# Autodesk Inventor assembly: ASSEMBLY_X_Axis_Carriage_and_Extruder_Belt_Gearbox
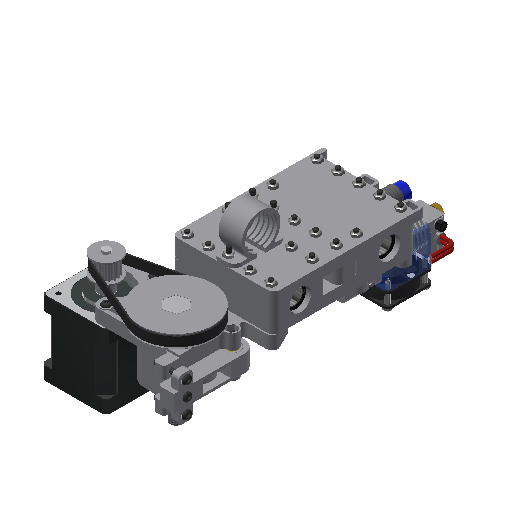
[picture p0: Inventor's stored thumbnail of the model, 512x512]
Saved by Autodesk Inventor 2026.1 (Build 301233000, 233)
## iProperties
Created: 2016-01-21
Part Number: ASSEMBLY_X_Axis_Carriage_and_Extruder_Belt_Gearbox
Material: Ogólny
Document SubType Name: Assembly
Designer: Andrzej
Author: Andrzej
## Documents named in this file (36)
- C:\Users\Andrzej\OneDrive\_DRIVE_SYNCH_FILES\__ BYTECHLAB PROJECTS\MECH - T-REX 300 – A completely new printer based on a old one\MCAD\1_REV1\ASSEMBLY_X_AXIS_CARRIAGE_AND_EXTRUDER\ASSEMBLY_X_Axis_Carriage_and_Extruder_Belt_Gearbox.iam
- C:\Users\Andrzej\OneDrive\_DRIVE_SYNCH_FILES\__ BYTECHLAB PROJECTS\MECH - T-REX 300 – A completely new printer based on a old one\MCAD\1_REV1\__COTS_PARTS\COTS_GENERIC_M8_Hobbed_Bolt.ipt
- C:\Users\Andrzej\OneDrive\_DRIVE_SYNCH_FILES\__ BYTECHLAB PROJECTS\MECH - T-REX 300 – A completely new printer based on a old one\MCAD\1_REV1\ASSEMBLY_X_AXIS_CARRIAGE_AND_EXTRUDER\3DP_ABS_HTD3M_Pulley_56_tooth_6mm.ipt
- C:\Users\Andrzej\OneDrive\_DRIVE_SYNCH_FILES\__ BYTECHLAB PROJECTS\MECH - T-REX 300 – A completely new printer based on a old one\MCAD\1_REV1\ASSEMBLY_X_AXIS_CARRIAGE_AND_EXTRUDER\3DP_ABS_X_Axis_Carriage_Front.ipt
- C:\Users\Andrzej\OneDrive\_DRIVE_SYNCH_FILES\__ BYTECHLAB PROJECTS\MECH - T-REX 300 – A completely new printer based on a old one\MCAD\1_REV1\ASSEMBLY_X_AXIS_CARRIAGE_AND_EXTRUDER\3DP_ABS_X_Axis_Carriage_Back.ipt
- C:\Users\Andrzej\OneDrive\_DRIVE_SYNCH_FILES\__ BYTECHLAB PROJECTS\MECH - T-REX 300 – A completely new printer based on a old one\MCAD\1_REV1\ASSEMBLY_X_AXIS_CARRIAGE_AND_EXTRUDER\3DP_ABS_Extruder_Body.ipt
- C:\Users\Andrzej\OneDrive\_DRIVE_SYNCH_FILES\__ BYTECHLAB PROJECTS\MECH - T-REX 300 – A completely new printer based on a old one\MCAD\1_REV1\ASSEMBLY_X_AXIS_CARRIAGE_AND_EXTRUDER\3DP_ABS_Extruder_Tensioning_Arm.ipt
- C:\Users\Andrzej\OneDrive\_DRIVE_SYNCH_FILES\__ BYTECHLAB PROJECTS\MECH - T-REX 300 – A completely new printer based on a old one\MCAD\1_REV1\ASSEMBLY_X_AXIS_CARRIAGE_AND_EXTRUDER\3DP_ABS_Extruder_Tensioning_Arm_Screw_Mount.ipt
- C:\Users\Andrzej\OneDrive\_DRIVE_SYNCH_FILES\__ BYTECHLAB PROJECTS\MECH - T-REX 300 – A completely new printer based on a old one\MCAD\1_REV1\ASSEMBLY_X_AXIS_CARRIAGE_AND_EXTRUDER\3DP_ABS_E3DV6_Mount.ipt
- C:\Users\Andrzej\OneDrive\_DRIVE_SYNCH_FILES\__ BYTECHLAB PROJECTS\MECH - T-REX 300 – A completely new printer based on a old one\MCAD\1_REV1\ASSEMBLY_X_AXIS_CARRIAGE_AND_EXTRUDER\CUT_PTFE_Tube_85mm.ipt
- C:\Users\Andrzej\OneDrive\_DRIVE_SYNCH_FILES\__ BYTECHLAB PROJECTS\MECH - T-REX 300 – A completely new printer based on a old one\MCAD\1_REV1\ASSEMBLY_X_AXIS_CARRIAGE_AND_EXTRUDER\3DP_ABS_Cable_Pipe_Mount.ipt
- C:\Users\Andrzej\OneDrive\_DRIVE_SYNCH_FILES\__ BYTECHLAB PROJECTS\MECH - T-REX 300 – A completely new printer based on a old one\MCAD\1_REV1\ASSEMBLY_X_AXIS_CARRIAGE_AND_EXTRUDER\3DP_ABS_PTFE_Tube_Stiffener.ipt
- C:\Users\Andrzej\OneDrive\_DRIVE_SYNCH_FILES\__ BYTECHLAB PROJECTS\MECH - T-REX 300 – A completely new printer based on a old one\MCAD\1_REV1\ASSEMBLY_X_AXIS_CARRIAGE_AND_EXTRUDER\3DP_ABS_E3DV6_Mounting_Clamp.ipt
- C:\Users\Andrzej\OneDrive\_DRIVE_SYNCH_FILES\__ BYTECHLAB PROJECTS\MECH - T-REX 300 – A completely new printer based on a old one\MCAD\1_REV1\__COTS_PARTS\COTS_E3D_V6_Hotend\COTS_E3D_V6_Hotend.iam
- C:\Users\Andrzej\OneDrive\_DRIVE_SYNCH_FILES\__ BYTECHLAB PROJECTS\MECH - T-REX 300 – A completely new printer based on a old one\MCAD\1_REV1\__COTS_PARTS\COTS_GENERIC_Induction_Distance_Sensor.ipt
- C:\Users\Andrzej\OneDrive\_DRIVE_SYNCH_FILES\__ BYTECHLAB PROJECTS\MECH - T-REX 300 – A completely new printer based on a old one\MCAD\1_REV1\ASSEMBLY_X_AXIS_CARRIAGE_AND_EXTRUDER\3DP_ABS_Induction_Sensor_Mount.ipt
- C:\Users\Andrzej\OneDrive\_DRIVE_SYNCH_FILES\__ BYTECHLAB PROJECTS\MECH - T-REX 300 – A completely new printer based on a old one\MCAD\1_REV1\ASSEMBLY_X_AXIS_CARRIAGE_AND_EXTRUDER\3DP_ABS_Induction_Sensor_Mounting_Clamp.ipt
- C:\Users\Andrzej\OneDrive\_DRIVE_SYNCH_FILES\__ BYTECHLAB PROJECTS\MECH - T-REX 300 – A completely new printer based on a old one\MCAD\1_REV1\ASSEMBLY_X_AXIS_CARRIAGE_AND_EXTRUDER\3DP_ABS_Induction_Sensor_Mount_Spacer.ipt
- C:\Users\Andrzej\OneDrive\_DRIVE_SYNCH_FILES\__ BYTECHLAB PROJECTS\MECH - T-REX 300 – A completely new printer based on a old one\MCAD\1_REV1\__COTS_PARTS\COTS_GENERIC_LM10UU_10mm_Linear_Bearing.ipt
- C:\Users\Andrzej\OneDrive\_DRIVE_SYNCH_FILES\__ BYTECHLAB PROJECTS\MECH - T-REX 300 – A completely new printer based on a old one\MCAD\1_REV1\__CONTENT_CENTER_PARTS\en-US\ISO 7380-1\ISO 7380-1 - M3 x 25.ipt
- C:\Users\Andrzej\OneDrive\_DRIVE_SYNCH_FILES\__ BYTECHLAB PROJECTS\MECH - T-REX 300 – A completely new printer based on a old one\MCAD\1_REV1\__CONTENT_CENTER_PARTS\en-US\DIN 934\DIN 934 - M3 x 0,5.ipt
- C:\Users\Andrzej\OneDrive\_DRIVE_SYNCH_FILES\__ BYTECHLAB PROJECTS\MECH - T-REX 300 – A completely new printer based on a old one\MCAD\1_REV1\__CONTENT_CENTER_PARTS\en-US\ISO 7380-1\ISO 7380-1 - M3 x 30.ipt
- C:\Users\Andrzej\OneDrive\_DRIVE_SYNCH_FILES\__ BYTECHLAB PROJECTS\MECH - T-REX 300 – A completely new printer based on a old one\MCAD\1_REV1\__CONTENT_CENTER_PARTS\en-US\ISO 7380-1\ISO 7380-1 - M3 x 20.ipt
- C:\Users\Andrzej\OneDrive\_DRIVE_SYNCH_FILES\__ BYTECHLAB PROJECTS\MECH - T-REX 300 – A completely new printer based on a old one\MCAD\1_REV1\__COTS_PARTS\COTS_GENERIC_ISO7380_M3x35.ipt
- C:\Users\Andrzej\OneDrive\_DRIVE_SYNCH_FILES\__ BYTECHLAB PROJECTS\MECH - T-REX 300 – A completely new printer based on a old one\MCAD\1_REV1\__COTS_PARTS\COTS_GENERIC_ISO7380_M3x45.ipt
- C:\Users\Andrzej\OneDrive\_DRIVE_SYNCH_FILES\__ BYTECHLAB PROJECTS\MECH - T-REX 300 – A completely new printer based on a old one\MCAD\1_REV1\__CONTENT_CENTER_PARTS\en-US\DIN 125-1  A\DIN 125 - A 3,2.ipt
- C:\Users\Andrzej\OneDrive\_DRIVE_SYNCH_FILES\__ BYTECHLAB PROJECTS\MECH - T-REX 300 – A completely new printer based on a old one\MCAD\1_REV1\__CONTENT_CENTER_PARTS\en-US\ISO 7380-1\ISO 7380-1 - M3 x 12.ipt
- C:\Users\Andrzej\OneDrive\_DRIVE_SYNCH_FILES\__ BYTECHLAB PROJECTS\MECH - T-REX 300 – A completely new printer based on a old one\MCAD\1_REV1\__CONTENT_CENTER_PARTS\en-US\DIN 934\DIN 934 - M8 x 1,25.ipt
- C:\Users\Andrzej\OneDrive\_DRIVE_SYNCH_FILES\__ BYTECHLAB PROJECTS\MECH - T-REX 300 – A completely new printer based on a old one\MCAD\1_REV1\__COTS_PARTS\COTS_GENERIC_608_2RS_8x22x7mm_bearing.ipt
- C:\Users\Andrzej\OneDrive\_DRIVE_SYNCH_FILES\__ BYTECHLAB PROJECTS\MECH - T-REX 300 – A completely new printer based on a old one\MCAD\1_REV1\__COTS_PARTS\COTS_GENERIC_623_ZZ_3x10x4mm_bearing\COTS_GENERIC_623_ZZ_3x10x4mm_bearing.ipt
- C:\Users\Andrzej\OneDrive\_DRIVE_SYNCH_FILES\__ BYTECHLAB PROJECTS\MECH - T-REX 300 – A completely new printer based on a old one\MCAD\1_REV1\__COTS_PARTS\COTS_Optibelt_Omega_HTD3M_204T_6mm.ipt
- C:\Users\Andrzej\OneDrive\_DRIVE_SYNCH_FILES\__ BYTECHLAB PROJECTS\MECH - T-REX 300 – A completely new printer based on a old one\MCAD\1_REV1\__COTS_PARTS\COTS_UNKNOWN_HTD3M_16T_Pulley\COTS_UNKNOWN_HTD3M_16T_Pulley.ipt
- C:\Users\Andrzej\OneDrive\_DRIVE_SYNCH_FILES\__ BYTECHLAB PROJECTS\MECH - T-REX 300 – A completely new printer based on a old one\MCAD\1_REV1\__COTS_PARTS\COTS_GENERIC_635_HZZ_5x19x6mm_bearing\COTS_GENERIC_635_HZZ_5x19x6mm_bearing.ipt
- C:\Users\Andrzej\OneDrive\_DRIVE_SYNCH_FILES\__ BYTECHLAB PROJECTS\MECH - T-REX 300 – A completely new printer based on a old one\MCAD\1_REV1\ASSEMBLY_X_AXIS_CARRIAGE_AND_EXTRUDER\CUT_STEEL_5x11mm_Rod.ipt
- C:\Users\Andrzej\OneDrive\_DRIVE_SYNCH_FILES\__ BYTECHLAB PROJECTS\MECH - T-REX 300 – A completely new printer based on a old one\MCAD\1_REV1\__COTS_PARTS\COTS_GENERIC_NEMA17_25mm_shaft.ipt
- C:\Users\Andrzej\OneDrive\_DRIVE_SYNCH_FILES\__ BYTECHLAB PROJECTS\MECH - T-REX 300 – A completely new printer based on a old one\MCAD\1_REV1\ASSEMBLY_X_AXIS_CARRIAGE_AND_EXTRUDER\3DP_ABS_Hobbed_Bolt_Spacer.ipt
## Components (100 placed, 35 different names)
1. 3DP_ABS_X_Axis_Carriage_Front:1 — Zestawiający:1, Równoległy:1, Równoległy:2, Zestawiający:2, Styczny:1, Zestawiający:19, Zestawiający:28, Mate:33, Mate:34, Mate:35, Mate:43, Mate:44, Mate:45, Mate:46, Mate:49, Mate:50, Mate:65, Mate:108, Mate:109, Mate:110, Mate:111, Mate:112, Mate:113, Mate:114, Mate:115, Mate:116, Mate:117, Mate:118, Mate:119, Mate:120, Mate:122, Mate:124, Mate:126, Mate:128, Mate:130, Mate:134, Mate:135, Mate:136
2. 3DP_ABS_X_Axis_Carriage_Back:1 — Zestawiający:1, Równoległy:1, Równoległy:2, Zestawiający:27, Mate:70, Mate:72, Mate:75, Mate:77, Mate:78, Mate:79, Mate:80, Mate:81, Mate:99, Mate:101, Mate:103, Mate:105, Mate:106, Mate:107, Mate:121, Mate:123, Mate:125, Mate:127, Mate:129, Mate:131, Mate:143, Mate:145, Insert:3, Insert:4, Insert:5, Insert:6
3. 3DP_ABS_Extruder_Body:1 — Zestawiający:2, Styczny:1, Zestawiający:4, Styczny:4, Zestawiający:6, Równoległy:3, Zestawiający:8, Wstaw:1, Mate:51, Mate:52, Mate:55, Mate:56, Mate:90, Mate:91, Mate:92, Mate:93, Mate:94, Mate:95, Mate:96, Mate:97, Mate:98, Mate:100, Mate:102, Mate:104, Mate:132, Mate:133, Mate:155, Mate:157, Mate:159, Mate:168, Mate:169, Mate:170, Mate:171, Angle:3, Mate:180, Mate:182, Mate:184, Mate:185, Mate:186, Mate:187
4. 3DP_ABS_HTD3M_Pulley_56_tooth_6mm:1 — Zestawiający:3, Styczny:2, Zestawiający:4, Angle:2, Mate:173, Mate:174, Mate:176
5. COTS_GENERIC_M8_Hobbed_Bolt:1 — Zestawiający:3, Styczny:2, Mate:53, Angle:2, Mate:188
6. COTS_GENERIC_NEMA17_25mm_shaft:1 — Zestawiający:6, Równoległy:3, Mate:154, Mate:156, Mate:158, Mate:172
7. 3DP_ABS_Extruder_Tensioning_Arm:1 — Styczny:4, Zestawiający:8, Zestawiający:9, Zestawiający:10, Równoległy:4, Mate:163, Mate:164, Mate:165, Mate:166, Mate:167, Mate:177, Mate:178, Mate:179, Flush:16
8. 3DP_ABS_Extruder_Tensioning_Arm_Screw_Mount:1 — Zestawiający:9, Zestawiający:10, Równoległy:4, Mate:160, Mate:161, Mate:162, Angle:3, Mate:181, Mate:183
9. 3DP_ABS_E3DV6_Mount:1 — Zestawiający:19, Zestawiający:30, Zestawiający:31, Zestawiający:32, Równoległy:13, Równoległy:14, Mate:57, Mate:58, Mate:60, Mate:61, Mate:65, Mate:66, Mate:67, Mate:68, Mate:69, Mate:71, Mate:73, Mate:74, Mate:76
10. CUT_PTFE_Tube_85mm:1 — Wstaw:1, Zestawiający:29
11. 3DP_ABS_Cable_Pipe_Mount:1 — Zestawiający:27, Mate:106, Mate:107, Insert:2, Mate:137
12. 3DP_ABS_PTFE_Tube_Stiffener:1 — Zestawiający:28, Zestawiający:29, Mate:138, Mate:139, Mate:140, Mate:141, Mate:142, Mate:144
13. 3DP_ABS_E3DV6_Mounting_Clamp:1 — Zestawiający:32, Równoległy:13, Równoległy:14, Mate:59, Mate:62, Mate:63, Mate:64
14. COTS_E3D_V6_Hotend:1 [sub-assembly] — Zestawiający:30, Zestawiający:31, Flush:15
15. COTS_GENERIC_Induction_Distance_Sensor:1 — Mate:40, Flush:15, Mate:41
16. 3DP_ABS_Induction_Sensor_Mount:1 — Mate:36, Mate:37, Mate:38, Mate:39, Mate:40, Angle:1, Mate:42, Mate:87, Mate:89, Mate:146, Mate:147, Mate:148, Mate:149, Mate:150, Mate:151, Mate:152, Mate:153
17. 3DP_ABS_Induction_Sensor_Mounting_Clamp:1 — Mate:41, Angle:1, Mate:42, Mate:82, Mate:83, Mate:84, Mate:85, Mate:86, Mate:88
18. 3DP_ABS_Induction_Sensor_Mount_Spacer:1 — Mate:33, Mate:34, Mate:35, Mate:36, Mate:37, Mate:38, Mate:39
19. COTS_GENERIC_LM10UU_10mm_Linear_Bearing:1 — Mate:45, Mate:48, Mate:49
20. COTS_GENERIC_LM10UU_10mm_Linear_Bearing:2 — Mate:46, Mate:48
21. COTS_GENERIC_LM10UU_10mm_Linear_Bearing:3 — Mate:44, Mate:47, Mate:50
22. COTS_GENERIC_LM10UU_10mm_Linear_Bearing:4 — Mate:43, Mate:47
23. COTS_GENERIC_608_2RS_8x22x7mm_bearing:1 — Mate:55, Mate:56, Mate:189
24. COTS_GENERIC_608_2RS_8x22x7mm_bearing:2 — Mate:51, Mate:52, Mate:53, Insert:10
25. COTS_GENERIC_623_ZZ_3x10x4mm_bearing:1 — Mate:165, Mate:166, Insert:12
26. COTS_GENERIC_623_ZZ_3x10x4mm_bearing:2 — Mate:164, Mate:167, Insert:11
27. COTS_Optibelt_Omega_HTD3M_204T_6mm:1 — Mate:174, Mate:175, Mate:176
28. COTS_UNKNOWN_HTD3M_16T_Pulley:1 — Mate:172, Mate:173, Mate:175
29. COTS_GENERIC_635_HZZ_5x19x6mm_bearing:1 — Mate:177, Mate:178
30. CUT_STEEL_5x11mm_Rod:1 — Mate:179, Flush:16
31. 3DP_ABS_Hobbed_Bolt_Spacer:1 — Mate:188, Mate:189
32. DIN 934 - replaced by DIN EN 24032/28673/28674 M3:30 — Mate:186, Mate:187
33. ISO 7380-1 M3 x 20:4 — Mate:182, Mate:183
34. DIN 934 - replaced by DIN EN 24032/28673/28674 M3:29 — Mate:184, Mate:185
35. ISO 7380-1 M3 x 20:3 — Mate:180, Mate:181
36. DIN 934 - replaced by DIN EN 24032/28673/28674 M3:28 — Mate:170, Mate:171
37. ISO 7380-1 M3 x 25:9 — Mate:168, Mate:169
38. DIN 125-1 A A 3,2:5 — Insert:12
39. DIN 125-1 A A 3,2:4 — Insert:11
40. DIN 934 - replaced by DIN EN 24032/28673/28674 M3:27 — Mate:162, Mate:163
41. ISO 7380-1 M3 x 12:4 — Mate:160, Mate:161
42. DIN 934 - replaced by DIN EN 24032/28673/28674 M8:1 — Insert:10
43. ISO 7380-1 M3 x 12:3 — Insert:9
44. ISO 7380-1 M3 x 12:2 — Insert:8
45. DIN 125-1 A A 3,2:3 — Mate:158, Mate:159, Insert:9
46. DIN 125-1 A A 3,2:2 — Mate:156, Mate:157, Insert:8
47. ISO 7380-1 M3 x 12:1 — Insert:7
48. DIN 125-1 A A 3,2:1 — Mate:154, Mate:155, Insert:7
49. DIN 934 - replaced by DIN EN 24032/28673/28674 M3:26 — Insert:6
50. DIN 934 - replaced by DIN EN 24032/28673/28674 M3:25 — Insert:5
51. DIN 934 - replaced by DIN EN 24032/28673/28674 M3:24 — Insert:4
52. DIN 934 - replaced by DIN EN 24032/28673/28674 M3:23 — Insert:3
53. COTS_GENERIC_ISO7380_M3x45:4 — Mate:148, Mate:153
54. COTS_GENERIC_ISO7380_M3x45:3 — Mate:149, Mate:151
55. COTS_GENERIC_ISO7380_M3x45:2 — Mate:147, Mate:152
56. COTS_GENERIC_ISO7380_M3x45:1 — Mate:146, Mate:150
57. DIN 934 - replaced by DIN EN 24032/28673/28674 M3:22 — Mate:144, Mate:145
58. ISO 7380-1 M3 x 30:11 — Mate:140, Mate:141
59. DIN 934 - replaced by DIN EN 24032/28673/28674 M3:21 — Mate:142, Mate:143
60. ISO 7380-1 M3 x 30:10 — Mate:138, Mate:139
61. DIN 934 - replaced by DIN EN 24032/28673/28674 M3:20 — Mate:136, Mate:137
62. ISO 7380-1 M3 x 30:9 — Mate:134, Mate:135
63. DIN 934 - replaced by DIN EN 24032/28673/28674 M3:19 — Insert:2
64. COTS_GENERIC_ISO7380_M3x35:2 — Mate:132, Mate:133
65. DIN 934 - replaced by DIN EN 24032/28673/28674 M3:18 — Mate:130, Mate:131
66. DIN 934 - replaced by DIN EN 24032/28673/28674 M3:17 — Mate:128, Mate:129
67. DIN 934 - replaced by DIN EN 24032/28673/28674 M3:16 — Mate:126, Mate:127
68. DIN 934 - replaced by DIN EN 24032/28673/28674 M3:15 — Mate:124, Mate:125
69. DIN 934 - replaced by DIN EN 24032/28673/28674 M3:14 — Mate:122, Mate:123
70. ISO 7380-1 M3 x 25:8 — Mate:118, Mate:119
71. ISO 7380-1 M3 x 25:7 — Mate:116, Mate:117
72. ISO 7380-1 M3 x 25:6 — Mate:114, Mate:115
73. ISO 7380-1 M3 x 25:5 — Mate:112, Mate:113
74. ISO 7380-1 M3 x 25:4 — Mate:110, Mate:111
75. DIN 934 - replaced by DIN EN 24032/28673/28674 M3:13 — Mate:120, Mate:121
76. ISO 7380-1 M3 x 25:3 — Mate:108, Mate:109
77. DIN 934 - replaced by DIN EN 24032/28673/28674 M3:12 — Mate:104, Mate:105
78. DIN 934 - replaced by DIN EN 24032/28673/28674 M3:11 — Mate:102, Mate:103
79. DIN 934 - replaced by DIN EN 24032/28673/28674 M3:10 — Mate:100, Mate:101
80. ISO 7380-1 M3 x 30:8 — Mate:96, Mate:97
81. ISO 7380-1 M3 x 30:7 — Mate:94, Mate:95
82. ISO 7380-1 M3 x 30:6 — Mate:92, Mate:93
83. DIN 934 - replaced by DIN EN 24032/28673/28674 M3:9 — Mate:98, Mate:99
84. ISO 7380-1 M3 x 30:5 — Mate:90, Mate:91
85. DIN 934 - replaced by DIN EN 24032/28673/28674 M3:8 — Mate:88, Mate:89
86. ISO 7380-1 M3 x 20:2 — Mate:84, Mate:85
87. DIN 934 - replaced by DIN EN 24032/28673/28674 M3:7 — Mate:86, Mate:87
88. ISO 7380-1 M3 x 20:1 — Mate:82, Mate:83
89. DIN 934 - replaced by DIN EN 24032/28673/28674 M3:6 — Mate:80, Mate:81
90. DIN 934 - replaced by DIN EN 24032/28673/28674 M3:5 — Mate:78, Mate:79
91. DIN 934 - replaced by DIN EN 24032/28673/28674 M3:4 — Mate:76, Mate:77
92. ISO 7380-1 M3 x 30:4 — Mate:72, Mate:73
93. ISO 7380-1 M3 x 30:3 — Mate:70, Mate:71
94. ISO 7380-1 M3 x 30:2 — Mate:68, Mate:69
95. DIN 934 - replaced by DIN EN 24032/28673/28674 M3:3 — Mate:74, Mate:75
96. ISO 7380-1 M3 x 30:1 — Mate:66, Mate:67
97. DIN 934 - replaced by DIN EN 24032/28673/28674 M3:2 — Mate:63, Mate:64
98. ISO 7380-1 M3 x 25:2 — Mate:59, Mate:60
99. DIN 934 - replaced by DIN EN 24032/28673/28674 M3:1 — Mate:61, Mate:62
100. ISO 7380-1 M3 x 25:1 — Mate:57, Mate:58
## Relationships (197: Mate 171, Insert 12, Flush 8, Tangent 3, Angle 3)
- Zestawiający:1 [Mate]: 3DP_ABS_X_Axis_Carriage_Front:1 ↔ 3DP_ABS_X_Axis_Carriage_Back:1
- Równoległy:1 [Flush]: 3DP_ABS_X_Axis_Carriage_Front:1 ↔ 3DP_ABS_X_Axis_Carriage_Back:1
- Równoległy:2 [Flush]: 3DP_ABS_X_Axis_Carriage_Front:1 ↔ 3DP_ABS_X_Axis_Carriage_Back:1
- Zestawiający:2 [Mate]: 3DP_ABS_X_Axis_Carriage_Front:1 ↔ 3DP_ABS_Extruder_Body:1
- Styczny:1 [Tangent]: 3DP_ABS_X_Axis_Carriage_Front:1 ↔ 3DP_ABS_Extruder_Body:1
- Zestawiający:3 [Mate]: 3DP_ABS_HTD3M_Pulley_56_tooth_6mm:1 ↔ COTS_GENERIC_M8_Hobbed_Bolt:1
- Styczny:2 [Tangent]: 3DP_ABS_HTD3M_Pulley_56_tooth_6mm:1 ↔ COTS_GENERIC_M8_Hobbed_Bolt:1
- Zestawiający:4 [Mate] (4 mm): 3DP_ABS_Extruder_Body:1 ↔ 3DP_ABS_HTD3M_Pulley_56_tooth_6mm:1
- Styczny:4 [Tangent]: 3DP_ABS_Extruder_Body:1 ↔ 3DP_ABS_Extruder_Tensioning_Arm:1
- Zestawiający:6 [Mate]: 3DP_ABS_Extruder_Body:1 ↔ COTS_GENERIC_NEMA17_25mm_shaft:1
- Równoległy:3 [Flush] (-1.5 mm): 3DP_ABS_Extruder_Body:1 ↔ COTS_GENERIC_NEMA17_25mm_shaft:1
- Zestawiający:8 [Mate] (0.5 mm): 3DP_ABS_Extruder_Body:1 ↔ 3DP_ABS_Extruder_Tensioning_Arm:1
- Zestawiający:9 [Mate]: 3DP_ABS_Extruder_Tensioning_Arm:1 ↔ 3DP_ABS_Extruder_Tensioning_Arm_Screw_Mount:1
- Zestawiający:10 [Mate]: 3DP_ABS_Extruder_Tensioning_Arm:1 ↔ 3DP_ABS_Extruder_Tensioning_Arm_Screw_Mount:1
- Równoległy:4 [Flush]: 3DP_ABS_Extruder_Tensioning_Arm:1 ↔ 3DP_ABS_Extruder_Tensioning_Arm_Screw_Mount:1
- Zestawiający:19 [Mate]: 3DP_ABS_X_Axis_Carriage_Front:1 ↔ 3DP_ABS_E3DV6_Mount:1
- Wstaw:1 [Insert]: 3DP_ABS_Extruder_Body:1 ↔ CUT_PTFE_Tube_85mm:1
- Zestawiający:27 [Mate]: 3DP_ABS_X_Axis_Carriage_Back:1 ↔ 3DP_ABS_Cable_Pipe_Mount:1
- Zestawiający:28 [Mate]: 3DP_ABS_X_Axis_Carriage_Front:1 ↔ 3DP_ABS_PTFE_Tube_Stiffener:1
- Zestawiający:29 [Mate]: CUT_PTFE_Tube_85mm:1 ↔ 3DP_ABS_PTFE_Tube_Stiffener:1
- Zestawiający:30 [Mate]: 3DP_ABS_E3DV6_Mount:1 ↔ COTS_E3D_V6_Hotend:1
- Zestawiający:31 [Mate] (0.2 mm): 3DP_ABS_E3DV6_Mount:1 ↔ COTS_E3D_V6_Hotend:1
- Zestawiający:32 [Mate]: 3DP_ABS_E3DV6_Mount:1 ↔ 3DP_ABS_E3DV6_Mounting_Clamp:1
- Równoległy:13 [Flush]: 3DP_ABS_E3DV6_Mount:1 ↔ 3DP_ABS_E3DV6_Mounting_Clamp:1
- Równoległy:14 [Flush]: 3DP_ABS_E3DV6_Mount:1 ↔ 3DP_ABS_E3DV6_Mounting_Clamp:1
- Mate:33: 3DP_ABS_X_Axis_Carriage_Front:1 ↔ 3DP_ABS_Induction_Sensor_Mount_Spacer:1
- Mate:34: 3DP_ABS_X_Axis_Carriage_Front:1 ↔ 3DP_ABS_Induction_Sensor_Mount_Spacer:1
- Mate:35: 3DP_ABS_X_Axis_Carriage_Front:1 ↔ 3DP_ABS_Induction_Sensor_Mount_Spacer:1
- Mate:36: 3DP_ABS_Induction_Sensor_Mount:1 ↔ 3DP_ABS_Induction_Sensor_Mount_Spacer:1
- Mate:37: 3DP_ABS_Induction_Sensor_Mount:1 ↔ 3DP_ABS_Induction_Sensor_Mount_Spacer:1
- Mate:38: 3DP_ABS_Induction_Sensor_Mount:1 ↔ 3DP_ABS_Induction_Sensor_Mount_Spacer:1
- Mate:39: 3DP_ABS_Induction_Sensor_Mount:1 ↔ 3DP_ABS_Induction_Sensor_Mount_Spacer:1
- Mate:40: COTS_GENERIC_Induction_Distance_Sensor:1 ↔ 3DP_ABS_Induction_Sensor_Mount:1
- Flush:15 (2 mm): COTS_E3D_V6_Hotend:1 ↔ COTS_GENERIC_Induction_Distance_Sensor:1
- Mate:41: COTS_GENERIC_Induction_Distance_Sensor:1 ↔ 3DP_ABS_Induction_Sensor_Mounting_Clamp:1
- Angle:1 (0 deg): 3DP_ABS_Induction_Sensor_Mount:1 ↔ 3DP_ABS_Induction_Sensor_Mounting_Clamp:1
- Mate:42: 3DP_ABS_Induction_Sensor_Mount:1 ↔ 3DP_ABS_Induction_Sensor_Mounting_Clamp:1
- Mate:43: 3DP_ABS_X_Axis_Carriage_Front:1 ↔ COTS_GENERIC_LM10UU_10mm_Linear_Bearing:4
- Mate:44: 3DP_ABS_X_Axis_Carriage_Front:1 ↔ COTS_GENERIC_LM10UU_10mm_Linear_Bearing:3
- Mate:45: 3DP_ABS_X_Axis_Carriage_Front:1 ↔ COTS_GENERIC_LM10UU_10mm_Linear_Bearing:1
- Mate:46: 3DP_ABS_X_Axis_Carriage_Front:1 ↔ COTS_GENERIC_LM10UU_10mm_Linear_Bearing:2
- Mate:47: COTS_GENERIC_LM10UU_10mm_Linear_Bearing:3 ↔ COTS_GENERIC_LM10UU_10mm_Linear_Bearing:4
- Mate:48: COTS_GENERIC_LM10UU_10mm_Linear_Bearing:1 ↔ COTS_GENERIC_LM10UU_10mm_Linear_Bearing:2
- Mate:49 (0.7 mm): 3DP_ABS_X_Axis_Carriage_Front:1 ↔ COTS_GENERIC_LM10UU_10mm_Linear_Bearing:1
- Mate:50 (0.7 mm): 3DP_ABS_X_Axis_Carriage_Front:1 ↔ COTS_GENERIC_LM10UU_10mm_Linear_Bearing:3
- Mate:51: 3DP_ABS_Extruder_Body:1 ↔ COTS_GENERIC_608_2RS_8x22x7mm_bearing:2
- Mate:52: 3DP_ABS_Extruder_Body:1 ↔ COTS_GENERIC_608_2RS_8x22x7mm_bearing:2
- Mate:53: COTS_GENERIC_M8_Hobbed_Bolt:1 ↔ COTS_GENERIC_608_2RS_8x22x7mm_bearing:2
- Mate:55: 3DP_ABS_Extruder_Body:1 ↔ COTS_GENERIC_608_2RS_8x22x7mm_bearing:1
- Mate:56: 3DP_ABS_Extruder_Body:1 ↔ COTS_GENERIC_608_2RS_8x22x7mm_bearing:1
- Angle:2 (0 deg): 3DP_ABS_HTD3M_Pulley_56_tooth_6mm:1 ↔ COTS_GENERIC_M8_Hobbed_Bolt:1
- Mate:57: 3DP_ABS_E3DV6_Mount:1 ↔ ISO 7380-1 M3 x 25:1
- Mate:58: 3DP_ABS_E3DV6_Mount:1 ↔ ISO 7380-1 M3 x 25:1
- Mate:59: 3DP_ABS_E3DV6_Mounting_Clamp:1 ↔ ISO 7380-1 M3 x 25:2
- Mate:60: 3DP_ABS_E3DV6_Mount:1 ↔ ISO 7380-1 M3 x 25:2
- Mate:61: 3DP_ABS_E3DV6_Mount:1 ↔ DIN 934 - replaced by DIN EN 24032/28673/28674 M3:1
- Mate:62: 3DP_ABS_E3DV6_Mounting_Clamp:1 ↔ DIN 934 - replaced by DIN EN 24032/28673/28674 M3:1
- Mate:63: 3DP_ABS_E3DV6_Mounting_Clamp:1 ↔ DIN 934 - replaced by DIN EN 24032/28673/28674 M3:2
- Mate:64: 3DP_ABS_E3DV6_Mounting_Clamp:1 ↔ DIN 934 - replaced by DIN EN 24032/28673/28674 M3:2
- Mate:65: 3DP_ABS_X_Axis_Carriage_Front:1 ↔ 3DP_ABS_E3DV6_Mount:1
- Mate:66: 3DP_ABS_E3DV6_Mount:1 ↔ ISO 7380-1 M3 x 30:1
- Mate:67: 3DP_ABS_E3DV6_Mount:1 ↔ ISO 7380-1 M3 x 30:1
- Mate:68: 3DP_ABS_E3DV6_Mount:1 ↔ ISO 7380-1 M3 x 30:2
- Mate:69: 3DP_ABS_E3DV6_Mount:1 ↔ ISO 7380-1 M3 x 30:2
- Mate:70: 3DP_ABS_X_Axis_Carriage_Back:1 ↔ ISO 7380-1 M3 x 30:3
- Mate:71: 3DP_ABS_E3DV6_Mount:1 ↔ ISO 7380-1 M3 x 30:3
- Mate:72: 3DP_ABS_X_Axis_Carriage_Back:1 ↔ ISO 7380-1 M3 x 30:4
- Mate:73: 3DP_ABS_E3DV6_Mount:1 ↔ ISO 7380-1 M3 x 30:4
- Mate:74: 3DP_ABS_E3DV6_Mount:1 ↔ DIN 934 - replaced by DIN EN 24032/28673/28674 M3:3
- Mate:75: 3DP_ABS_X_Axis_Carriage_Back:1 ↔ DIN 934 - replaced by DIN EN 24032/28673/28674 M3:3
- Mate:76: 3DP_ABS_E3DV6_Mount:1 ↔ DIN 934 - replaced by DIN EN 24032/28673/28674 M3:4
- Mate:77: 3DP_ABS_X_Axis_Carriage_Back:1 ↔ DIN 934 - replaced by DIN EN 24032/28673/28674 M3:4
- Mate:78: 3DP_ABS_X_Axis_Carriage_Back:1 ↔ DIN 934 - replaced by DIN EN 24032/28673/28674 M3:5
- Mate:79: 3DP_ABS_X_Axis_Carriage_Back:1 ↔ DIN 934 - replaced by DIN EN 24032/28673/28674 M3:5
- Mate:80: 3DP_ABS_X_Axis_Carriage_Back:1 ↔ DIN 934 - replaced by DIN EN 24032/28673/28674 M3:6
- Mate:81: 3DP_ABS_X_Axis_Carriage_Back:1 ↔ DIN 934 - replaced by DIN EN 24032/28673/28674 M3:6
- Mate:82: 3DP_ABS_Induction_Sensor_Mounting_Clamp:1 ↔ ISO 7380-1 M3 x 20:1
- Mate:83: 3DP_ABS_Induction_Sensor_Mounting_Clamp:1 ↔ ISO 7380-1 M3 x 20:1
- Mate:84: 3DP_ABS_Induction_Sensor_Mounting_Clamp:1 ↔ ISO 7380-1 M3 x 20:2
- Mate:85: 3DP_ABS_Induction_Sensor_Mounting_Clamp:1 ↔ ISO 7380-1 M3 x 20:2
- Mate:86: 3DP_ABS_Induction_Sensor_Mounting_Clamp:1 ↔ DIN 934 - replaced by DIN EN 24032/28673/28674 M3:7
- Mate:87: 3DP_ABS_Induction_Sensor_Mount:1 ↔ DIN 934 - replaced by DIN EN 24032/28673/28674 M3:7
- Mate:88: 3DP_ABS_Induction_Sensor_Mounting_Clamp:1 ↔ DIN 934 - replaced by DIN EN 24032/28673/28674 M3:8
- Mate:89: 3DP_ABS_Induction_Sensor_Mount:1 ↔ DIN 934 - replaced by DIN EN 24032/28673/28674 M3:8
- Mate:90: 3DP_ABS_Extruder_Body:1 ↔ ISO 7380-1 M3 x 30:5
- Mate:91: 3DP_ABS_Extruder_Body:1 ↔ ISO 7380-1 M3 x 30:5
- Mate:92: 3DP_ABS_Extruder_Body:1 ↔ ISO 7380-1 M3 x 30:6
- Mate:93: 3DP_ABS_Extruder_Body:1 ↔ ISO 7380-1 M3 x 30:6
- Mate:94: 3DP_ABS_Extruder_Body:1 ↔ ISO 7380-1 M3 x 30:7
- Mate:95: 3DP_ABS_Extruder_Body:1 ↔ ISO 7380-1 M3 x 30:7
- Mate:96: 3DP_ABS_Extruder_Body:1 ↔ ISO 7380-1 M3 x 30:8
- Mate:97: 3DP_ABS_Extruder_Body:1 ↔ ISO 7380-1 M3 x 30:8
- Mate:98: 3DP_ABS_Extruder_Body:1 ↔ DIN 934 - replaced by DIN EN 24032/28673/28674 M3:9
- Mate:99: 3DP_ABS_X_Axis_Carriage_Back:1 ↔ DIN 934 - replaced by DIN EN 24032/28673/28674 M3:9
- Mate:100: 3DP_ABS_Extruder_Body:1 ↔ DIN 934 - replaced by DIN EN 24032/28673/28674 M3:10
- Mate:101: 3DP_ABS_X_Axis_Carriage_Back:1 ↔ DIN 934 - replaced by DIN EN 24032/28673/28674 M3:10
- Mate:102: 3DP_ABS_Extruder_Body:1 ↔ DIN 934 - replaced by DIN EN 24032/28673/28674 M3:11
- Mate:103: 3DP_ABS_X_Axis_Carriage_Back:1 ↔ DIN 934 - replaced by DIN EN 24032/28673/28674 M3:11
- Mate:104: 3DP_ABS_Extruder_Body:1 ↔ DIN 934 - replaced by DIN EN 24032/28673/28674 M3:12
- Mate:105: 3DP_ABS_X_Axis_Carriage_Back:1 ↔ DIN 934 - replaced by DIN EN 24032/28673/28674 M3:12
- Mate:106: 3DP_ABS_X_Axis_Carriage_Back:1 ↔ 3DP_ABS_Cable_Pipe_Mount:1
- Mate:107: 3DP_ABS_X_Axis_Carriage_Back:1 ↔ 3DP_ABS_Cable_Pipe_Mount:1
- Mate:108: 3DP_ABS_X_Axis_Carriage_Front:1 ↔ ISO 7380-1 M3 x 25:3
- Mate:109: 3DP_ABS_X_Axis_Carriage_Front:1 ↔ ISO 7380-1 M3 x 25:3
- Mate:110: 3DP_ABS_X_Axis_Carriage_Front:1 ↔ ISO 7380-1 M3 x 25:4
- Mate:111: 3DP_ABS_X_Axis_Carriage_Front:1 ↔ ISO 7380-1 M3 x 25:4
- Mate:112: 3DP_ABS_X_Axis_Carriage_Front:1 ↔ ISO 7380-1 M3 x 25:5
- Mate:113: 3DP_ABS_X_Axis_Carriage_Front:1 ↔ ISO 7380-1 M3 x 25:5
- Mate:114: 3DP_ABS_X_Axis_Carriage_Front:1 ↔ ISO 7380-1 M3 x 25:6
- Mate:115: 3DP_ABS_X_Axis_Carriage_Front:1 ↔ ISO 7380-1 M3 x 25:6
- Mate:116: 3DP_ABS_X_Axis_Carriage_Front:1 ↔ ISO 7380-1 M3 x 25:7
- Mate:117: 3DP_ABS_X_Axis_Carriage_Front:1 ↔ ISO 7380-1 M3 x 25:7
- Mate:118: 3DP_ABS_X_Axis_Carriage_Front:1 ↔ ISO 7380-1 M3 x 25:8
- Mate:119: 3DP_ABS_X_Axis_Carriage_Front:1 ↔ ISO 7380-1 M3 x 25:8
- Mate:120: 3DP_ABS_X_Axis_Carriage_Front:1 ↔ DIN 934 - replaced by DIN EN 24032/28673/28674 M3:13
- Mate:121: 3DP_ABS_X_Axis_Carriage_Back:1 ↔ DIN 934 - replaced by DIN EN 24032/28673/28674 M3:13
- Mate:122: 3DP_ABS_X_Axis_Carriage_Front:1 ↔ DIN 934 - replaced by DIN EN 24032/28673/28674 M3:14
- Mate:123: 3DP_ABS_X_Axis_Carriage_Back:1 ↔ DIN 934 - replaced by DIN EN 24032/28673/28674 M3:14
- Mate:124: 3DP_ABS_X_Axis_Carriage_Front:1 ↔ DIN 934 - replaced by DIN EN 24032/28673/28674 M3:15
- Mate:125: 3DP_ABS_X_Axis_Carriage_Back:1 ↔ DIN 934 - replaced by DIN EN 24032/28673/28674 M3:15
- Mate:126: 3DP_ABS_X_Axis_Carriage_Front:1 ↔ DIN 934 - replaced by DIN EN 24032/28673/28674 M3:16
- Mate:127: 3DP_ABS_X_Axis_Carriage_Back:1 ↔ DIN 934 - replaced by DIN EN 24032/28673/28674 M3:16
- Mate:128: 3DP_ABS_X_Axis_Carriage_Front:1 ↔ DIN 934 - replaced by DIN EN 24032/28673/28674 M3:17
- Mate:129: 3DP_ABS_X_Axis_Carriage_Back:1 ↔ DIN 934 - replaced by DIN EN 24032/28673/28674 M3:17
- Mate:130: 3DP_ABS_X_Axis_Carriage_Front:1 ↔ DIN 934 - replaced by DIN EN 24032/28673/28674 M3:18
- Mate:131: 3DP_ABS_X_Axis_Carriage_Back:1 ↔ DIN 934 - replaced by DIN EN 24032/28673/28674 M3:18
- Mate:132: 3DP_ABS_Extruder_Body:1 ↔ COTS_GENERIC_ISO7380_M3x35:2
- Mate:133: 3DP_ABS_Extruder_Body:1 ↔ COTS_GENERIC_ISO7380_M3x35:2
- Insert:2: 3DP_ABS_Cable_Pipe_Mount:1 ↔ DIN 934 - replaced by DIN EN 24032/28673/28674 M3:19
- Mate:134: 3DP_ABS_X_Axis_Carriage_Front:1 ↔ ISO 7380-1 M3 x 30:9
- Mate:135: 3DP_ABS_X_Axis_Carriage_Front:1 ↔ ISO 7380-1 M3 x 30:9
- Mate:136: 3DP_ABS_X_Axis_Carriage_Front:1 ↔ DIN 934 - replaced by DIN EN 24032/28673/28674 M3:20
- Mate:137: 3DP_ABS_Cable_Pipe_Mount:1 ↔ DIN 934 - replaced by DIN EN 24032/28673/28674 M3:20
- Mate:138: 3DP_ABS_PTFE_Tube_Stiffener:1 ↔ ISO 7380-1 M3 x 30:10
- Mate:139: 3DP_ABS_PTFE_Tube_Stiffener:1 ↔ ISO 7380-1 M3 x 30:10
- Mate:140: 3DP_ABS_PTFE_Tube_Stiffener:1 ↔ ISO 7380-1 M3 x 30:11
- Mate:141: 3DP_ABS_PTFE_Tube_Stiffener:1 ↔ ISO 7380-1 M3 x 30:11
- Mate:142: 3DP_ABS_PTFE_Tube_Stiffener:1 ↔ DIN 934 - replaced by DIN EN 24032/28673/28674 M3:21
- Mate:143: 3DP_ABS_X_Axis_Carriage_Back:1 ↔ DIN 934 - replaced by DIN EN 24032/28673/28674 M3:21
- Mate:144: 3DP_ABS_PTFE_Tube_Stiffener:1 ↔ DIN 934 - replaced by DIN EN 24032/28673/28674 M3:22
- Mate:145: 3DP_ABS_X_Axis_Carriage_Back:1 ↔ DIN 934 - replaced by DIN EN 24032/28673/28674 M3:22
- Mate:146: 3DP_ABS_Induction_Sensor_Mount:1 ↔ COTS_GENERIC_ISO7380_M3x45:1
- Mate:147: 3DP_ABS_Induction_Sensor_Mount:1 ↔ COTS_GENERIC_ISO7380_M3x45:2
- Mate:148: 3DP_ABS_Induction_Sensor_Mount:1 ↔ COTS_GENERIC_ISO7380_M3x45:4
- Mate:149: 3DP_ABS_Induction_Sensor_Mount:1 ↔ COTS_GENERIC_ISO7380_M3x45:3
- Mate:150: 3DP_ABS_Induction_Sensor_Mount:1 ↔ COTS_GENERIC_ISO7380_M3x45:1
- Mate:151: 3DP_ABS_Induction_Sensor_Mount:1 ↔ COTS_GENERIC_ISO7380_M3x45:3
- Mate:152: 3DP_ABS_Induction_Sensor_Mount:1 ↔ COTS_GENERIC_ISO7380_M3x45:2
- Mate:153: 3DP_ABS_Induction_Sensor_Mount:1 ↔ COTS_GENERIC_ISO7380_M3x45:4
- Insert:3: 3DP_ABS_X_Axis_Carriage_Back:1 ↔ DIN 934 - replaced by DIN EN 24032/28673/28674 M3:23
- Insert:4: 3DP_ABS_X_Axis_Carriage_Back:1 ↔ DIN 934 - replaced by DIN EN 24032/28673/28674 M3:24
- Insert:5: 3DP_ABS_X_Axis_Carriage_Back:1 ↔ DIN 934 - replaced by DIN EN 24032/28673/28674 M3:25
- Insert:6: 3DP_ABS_X_Axis_Carriage_Back:1 ↔ DIN 934 - replaced by DIN EN 24032/28673/28674 M3:26
- Mate:154: COTS_GENERIC_NEMA17_25mm_shaft:1 ↔ DIN 125-1 A A 3,2:1
- Mate:155: 3DP_ABS_Extruder_Body:1 ↔ DIN 125-1 A A 3,2:1
- Mate:156: COTS_GENERIC_NEMA17_25mm_shaft:1 ↔ DIN 125-1 A A 3,2:2
- Mate:157: 3DP_ABS_Extruder_Body:1 ↔ DIN 125-1 A A 3,2:2
- Mate:158: COTS_GENERIC_NEMA17_25mm_shaft:1 ↔ DIN 125-1 A A 3,2:3
- Mate:159: 3DP_ABS_Extruder_Body:1 ↔ DIN 125-1 A A 3,2:3
- Insert:7: ISO 7380-1 M3 x 12:1 ↔ DIN 125-1 A A 3,2:1
- Insert:8: ISO 7380-1 M3 x 12:2 ↔ DIN 125-1 A A 3,2:2
- Insert:9: ISO 7380-1 M3 x 12:3 ↔ DIN 125-1 A A 3,2:3
- Insert:10: COTS_GENERIC_608_2RS_8x22x7mm_bearing:2 ↔ DIN 934 - replaced by DIN EN 24032/28673/28674 M8:1
- Mate:160: 3DP_ABS_Extruder_Tensioning_Arm_Screw_Mount:1 ↔ ISO 7380-1 M3 x 12:4
- Mate:161: 3DP_ABS_Extruder_Tensioning_Arm_Screw_Mount:1 ↔ ISO 7380-1 M3 x 12:4
- Mate:162: 3DP_ABS_Extruder_Tensioning_Arm_Screw_Mount:1 ↔ DIN 934 - replaced by DIN EN 24032/28673/28674 M3:27
- Mate:163: 3DP_ABS_Extruder_Tensioning_Arm:1 ↔ DIN 934 - replaced by DIN EN 24032/28673/28674 M3:27
- Mate:164: 3DP_ABS_Extruder_Tensioning_Arm:1 ↔ COTS_GENERIC_623_ZZ_3x10x4mm_bearing:2
- Mate:165: 3DP_ABS_Extruder_Tensioning_Arm:1 ↔ COTS_GENERIC_623_ZZ_3x10x4mm_bearing:1
- Mate:166: 3DP_ABS_Extruder_Tensioning_Arm:1 ↔ COTS_GENERIC_623_ZZ_3x10x4mm_bearing:1
- Mate:167: 3DP_ABS_Extruder_Tensioning_Arm:1 ↔ COTS_GENERIC_623_ZZ_3x10x4mm_bearing:2
- Insert:11: COTS_GENERIC_623_ZZ_3x10x4mm_bearing:2 ↔ DIN 125-1 A A 3,2:4
- Insert:12: COTS_GENERIC_623_ZZ_3x10x4mm_bearing:1 ↔ DIN 125-1 A A 3,2:5
- Mate:168: 3DP_ABS_Extruder_Body:1 ↔ ISO 7380-1 M3 x 25:9
- Mate:169: 3DP_ABS_Extruder_Body:1 ↔ ISO 7380-1 M3 x 25:9
- Mate:170: 3DP_ABS_Extruder_Body:1 ↔ DIN 934 - replaced by DIN EN 24032/28673/28674 M3:28
- Mate:171: 3DP_ABS_Extruder_Body:1 ↔ DIN 934 - replaced by DIN EN 24032/28673/28674 M3:28
- Mate:172: COTS_GENERIC_NEMA17_25mm_shaft:1 ↔ COTS_UNKNOWN_HTD3M_16T_Pulley:1
- Mate:173 (1.25 mm): 3DP_ABS_HTD3M_Pulley_56_tooth_6mm:1 ↔ COTS_UNKNOWN_HTD3M_16T_Pulley:1
- Mate:174: 3DP_ABS_HTD3M_Pulley_56_tooth_6mm:1 ↔ COTS_Optibelt_Omega_HTD3M_204T_6mm:1
- Mate:175: COTS_Optibelt_Omega_HTD3M_204T_6mm:1 ↔ COTS_UNKNOWN_HTD3M_16T_Pulley:1
- Mate:176 (0.25 mm): 3DP_ABS_HTD3M_Pulley_56_tooth_6mm:1 ↔ COTS_Optibelt_Omega_HTD3M_204T_6mm:1
- Mate:177: 3DP_ABS_Extruder_Tensioning_Arm:1 ↔ COTS_GENERIC_635_HZZ_5x19x6mm_bearing:1
- Mate:178 (0.75 mm): 3DP_ABS_Extruder_Tensioning_Arm:1 ↔ COTS_GENERIC_635_HZZ_5x19x6mm_bearing:1
- Mate:179: 3DP_ABS_Extruder_Tensioning_Arm:1 ↔ CUT_STEEL_5x11mm_Rod:1
- Flush:16: 3DP_ABS_Extruder_Tensioning_Arm:1 ↔ CUT_STEEL_5x11mm_Rod:1
- Angle:3 (0 deg): 3DP_ABS_Extruder_Body:1 ↔ 3DP_ABS_Extruder_Tensioning_Arm_Screw_Mount:1
- Mate:180: 3DP_ABS_Extruder_Body:1 ↔ ISO 7380-1 M3 x 20:3
- Mate:181: 3DP_ABS_Extruder_Tensioning_Arm_Screw_Mount:1 ↔ ISO 7380-1 M3 x 20:3
- Mate:182: 3DP_ABS_Extruder_Body:1 ↔ ISO 7380-1 M3 x 20:4
- Mate:183: 3DP_ABS_Extruder_Tensioning_Arm_Screw_Mount:1 ↔ ISO 7380-1 M3 x 20:4
- Mate:184: 3DP_ABS_Extruder_Body:1 ↔ DIN 934 - replaced by DIN EN 24032/28673/28674 M3:29
- Mate:185: 3DP_ABS_Extruder_Body:1 ↔ DIN 934 - replaced by DIN EN 24032/28673/28674 M3:29
- Mate:186: 3DP_ABS_Extruder_Body:1 ↔ DIN 934 - replaced by DIN EN 24032/28673/28674 M3:30
- Mate:187: 3DP_ABS_Extruder_Body:1 ↔ DIN 934 - replaced by DIN EN 24032/28673/28674 M3:30
- Mate:188: COTS_GENERIC_M8_Hobbed_Bolt:1 ↔ 3DP_ABS_Hobbed_Bolt_Spacer:1
- Mate:189: COTS_GENERIC_608_2RS_8x22x7mm_bearing:1 ↔ 3DP_ABS_Hobbed_Bolt_Spacer:1
